# Autodesk Inventor assembly: Body_as
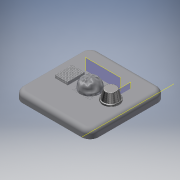
[picture p0: Inventor's stored thumbnail of the model, 180x180]
Saved by Autodesk Inventor 2017.2 (Build 212223000, 223)
## iProperties
Created: 2017-02-21
Part Number: Body_as
Document SubType Name: Assembly
Designer: prosp
Author: prosp
## Documents named in this file (6)
- C:\Users\prosp\OneDrive\Documents\Inventor\PROD_SmartUnit01\Body_as.iam
- C:\Users\prosp\OneDrive\Documents\Inventor\PROD_SmartUnit01\Body.ipt
- C:\Users\prosp\OneDrive\Documents\Inventor\PROD_SmartUnit01\MotionSensor.ipt
- C:\Users\prosp\OneDrive\Documents\Inventor\PROD_SmartUnit01\CO2_Sensor.ipt
- C:\Users\prosp\OneDrive\Documents\Inventor\PROD_SmartUnit01\DHT22.ipt
- C:\Users\prosp\OneDrive\Documents\Inventor\PROD_SmartUnit01\OLED_128x32.ipt
## Components (5 placed, 5 different names)
1. Body:1 — Mate:2, Mate:3, Mate:4, Mate:5, Mate:6, Mate:7, Mate:8, Mate:9, Mate:10, Mate:11, Mate:12, Mate:13, Flush:1, Flush:2, Mate:14, Mate:15
2. MotionSensor:1 — Mate:1, Mate:8, Mate:9, Mate:13, Flush:1, Flush:2
3. CO2_Sensor:1 — Mate:6, Mate:7, Mate:14
4. DHT22:1 — Mate:10, Mate:11, Mate:12
5. OLED_128x32:1 — Angle:1, Mate:2, Mate:3, Mate:4, Mate:5, Mate:15
## Relationships (18: Mate 15, Flush 2, Angle 1)
- Mate:1: MotionSensor:1
- Angle:1 (0 deg): OLED_128x32:1
- Mate:2 (11 mm): Body:1 ↔ OLED_128x32:1
- Mate:3 (9.5 mm): Body:1 ↔ OLED_128x32:1
- Mate:4 (9.5 mm): Body:1 ↔ OLED_128x32:1
- Mate:5 (24.5 mm): Body:1 ↔ OLED_128x32:1
- Mate:6 (9 mm): Body:1 ↔ CO2_Sensor:1
- Mate:7 (29.68 mm): Body:1 ↔ CO2_Sensor:1
- Mate:8 (27 mm): Body:1 ↔ MotionSensor:1
- Mate:9 (31.25 mm): Body:1 ↔ MotionSensor:1
- Mate:10 (33 mm): Body:1 ↔ DHT22:1
- Mate:11 (59.5 mm): Body:1 ↔ DHT22:1
- Mate:12 (1 mm): Body:1 ↔ DHT22:1
- Mate:13: Body:1 ↔ MotionSensor:1
- Flush:1: Body:1 ↔ MotionSensor:1
- Flush:2: Body:1 ↔ MotionSensor:1
- Mate:14 (1 mm): Body:1 ↔ CO2_Sensor:1
- Mate:15: Body:1 ↔ OLED_128x32:1
